# Autodesk Inventor assembly: OdroidAssembly
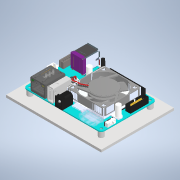
[picture p0: Inventor's stored thumbnail of the model, 180x180]
Saved by Autodesk Inventor 2020 (Build 240168000, 168)
## iProperties
Created: 2019-06-15
Part Number: OdroidAssembly
Document SubType Name: Assembly
Designer: amirt
Author: amirt
## Documents named in this file (4)
- C:\Users\amirt\Documents\Inventor\Drone\OdroidParts\OdroidAssembly.iam
- C:\Users\amirt\Documents\Inventor\Drone\Imported Components\Odroid-XU4 v1.ipt
- C:\Users\amirt\Documents\Inventor\Drone\3DPrint\odroidstandoff.ipt
- C:\Users\amirt\Documents\Inventor\Drone\3DPrint\BasePlate.ipt
## Components (6 placed, 3 different names)
1. Odroid-XU4 v1:1 — Flush:1, Flush:2, Mate:1, Insert:1, Mate:2, Mate:3
2. odroidstandoff:1 — Flush:1, Flush:2, Flush:3
3. odroidstandoff:2 — Mate:2
4. odroidstandoff:3 — Mate:1, Insert:1
5. odroidstandoff:4 — Mate:3
6. BasePlate:1 — Flush:3
## Relationships (7: Flush 3, Mate 3, Insert 1)
- Flush:1: Odroid-XU4 v1:1 ↔ odroidstandoff:1
- Flush:2: Odroid-XU4 v1:1 ↔ odroidstandoff:1
- Mate:1: Odroid-XU4 v1:1 ↔ odroidstandoff:3
- Insert:1: Odroid-XU4 v1:1 ↔ odroidstandoff:3
- Mate:2: Odroid-XU4 v1:1 ↔ odroidstandoff:2
- Mate:3: Odroid-XU4 v1:1 ↔ odroidstandoff:4
- Flush:3: odroidstandoff:1 ↔ BasePlate:1
